# Autodesk Inventor assembly: Air_Engine_ASM
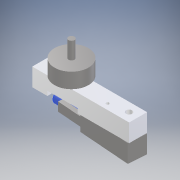
[picture p0: Inventor's stored thumbnail of the model, 180x180]
Saved by Autodesk Inventor 2018 (Build 220112000, 112)
## iProperties
Created: 2017-09-20
Part Number: Air_Engine_ASM
Document SubType Name: Assembly
Designer: Intel
Author: Intel
## Documents named in this file (8)
- C:\Users\Intel\Documents\Inventor\Air Engine\Air_Engine_ASM.iam
- C:\Users\Intel\Documents\Inventor\Air Engine\CrankShaft.ipt
- C:\Users\Intel\Documents\Inventor\Air Engine\Flywheel.ipt
- C:\Users\Intel\Documents\Inventor\Air Engine\Piston Block.ipt
- C:\Users\Intel\Documents\Inventor\Air Engine\Piston Bushing.ipt
- C:\Users\Intel\Documents\Inventor\Air Engine\Piston.ipt
- C:\Users\Intel\Documents\Inventor\Air Engine\Standard Bushing.ipt
- C:\Users\Intel\Documents\Inventor\Air Engine\Standard.ipt
## Components (7 placed, 7 different names)
1. CrankShaft:1 — Mate:7, Mate:8, Mate:9, Mate:10
2. Flywheel:1 — Mate:10, Mate:11
3. Piston Block:1 — Mate:2, Mate:3, Mate:16
4. Piston Bushing:1 — Mate:4, Mate:5, Mate:9
5. Piston:1 — Mate:4, Mate:5, Mate:16
6. Standard Bushing:1 — Mate:1, Flush:1, Mate:7
7. Standard:1 — Mate:1, Flush:1, Mate:2, Mate:3, Mate:8, Mate:11, Mate:12, Mate:13, Mate:15
## Relationships (15: Mate 14, Flush 1)
- Mate:1: Standard Bushing:1 ↔ Standard:1
- Flush:1: Standard Bushing:1 ↔ Standard:1
- Mate:2: Piston Block:1 ↔ Standard:1
- Mate:3: Piston Block:1 ↔ Standard:1
- Mate:4: Piston Bushing:1 ↔ Piston:1
- Mate:5: Piston Bushing:1 ↔ Piston:1
- Mate:7: CrankShaft:1 ↔ Standard Bushing:1
- Mate:8: CrankShaft:1 ↔ Standard:1
- Mate:9: CrankShaft:1 ↔ Piston Bushing:1
- Mate:10: CrankShaft:1 ↔ Flywheel:1
- Mate:11: Flywheel:1 ↔ Standard:1
- Mate:12: Standard:1
- Mate:13: Standard:1
- Mate:15: Standard:1
- Mate:16: Piston Block:1 ↔ Piston:1
